# Autodesk Inventor assembly: Horizontal Weapon Assembly (Type FD)
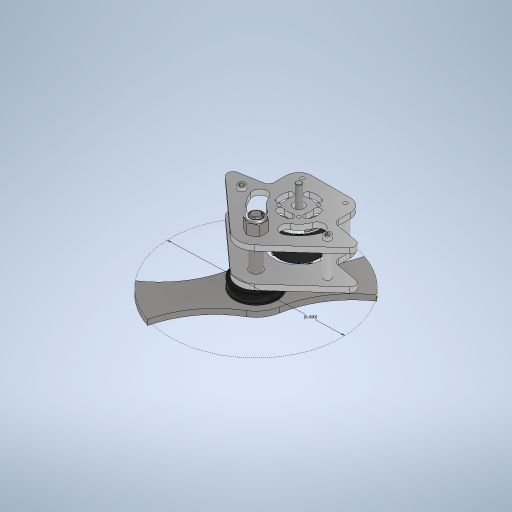
[picture p0: Inventor's stored thumbnail of the model, 512x512]
Saved by Autodesk Inventor 2023.2 (Build 272271000, 271)
## iProperties
Created: 2022-11-17
Part Number: Horizontal Weapon Assembly (Type FD)
Document SubType Name: Assembly
Designer: Nathan Cai
Mass: 397.62 g
Surface Area: 730.146 cm^2
Volume: 92.9751 cm^3
Density: 4.27663 g/cm^3
Author: Nathan Cai
## Documents named in this file (9)
- E:\Documents\Inventor\0.3rd Lawette - V3.5\Horizontal Weapon Assembly (Type FD)\Horizontal Weapon Assembly (Type FD).iam
- E:\Documents\Inventor\0.3rd Lawette - V3.5\Horizontal Weapon Assembly (Type FD)\Upright.ipt
- E:\Documents\Inventor\0.3rd Lawette - V3.5\Horizontal Weapon Assembly (Type FD)\Upright (Lower).ipt
- E:\Documents\Inventor\0.3rd Lawette - V3.5\Standoff 1in.ipt
- E:\Documents\Inventor\0.3rd Lawette - V3.5\Standoff 1.5in.ipt
- E:\Documents\Inventor\0.3rd Lawette - V3.5\Horizontal Weapon Assembly (Type FD)\90807A139_Same-Size Thread Alloy Steel Shoulder Screw.ipt
- E:\Documents\Inventor\0.3rd Lawette - V3.5\Horizontal Weapon Assembly (Type FD)\90630A121_High-Strength Steel Nylon-Insert Locknut.ipt
- E:\Documents\Inventor\0.3rd Lawette - V3.5\Horizontal Weapon Assembly (Type FD)\Weapon Stack.iam
- E:\Documents\Inventor\0.3rd Lawette - V3.5\Horizontal Weapon Assembly (Type FD)\Propdrive 3536\Propdrive V2 3536.iam
## Components (10 placed, 8 different names)
1. Upright:1 — Mate:4, Mate:5, Mate:6, Mate:7, Mate:8, Mate:9, Mate:10, Mate:11, Mate:12, Mate:13, Mate:14, Mate:16, Mate:19, Mate:20, Mate:21
2. Upright (Lower):1 — Mate:4, Mate:5, Mate:6, Flush:1, Flush:2
3. Standoff 1in:1 — Mate:7, Mate:10
4. Standoff 1in:2 — Mate:8, Mate:9
5. Standoff 1.5in:1 — Mate:11, Flush:1
6. Standoff 1.5in:2 — Mate:12, Flush:2
7. 90807A139_Same-Size Thread Alloy Steel Shoulder Screw:1 — Mate:13, Mate:14, Mate:15, Mate:17, Mate:18
8. 90630A121_High-Strength Steel Nylon-Insert Locknut:1 — Mate:15, Mate:16
9. Weapon Stack:1 [sub-assembly] — Mate:17, Mate:18
10. Propdrive V2 3536:1 [sub-assembly] — Mate:19, Mate:20, Mate:21
## Relationships (20: Mate 18, Flush 2)
- Mate:4: Upright:1 ↔ Upright (Lower):1
- Mate:5 (25.4 mm): Upright:1 ↔ Upright (Lower):1
- Mate:6: Upright:1 ↔ Upright (Lower):1
- Mate:7: Upright:1 ↔ Standoff 1in:1
- Mate:8: Upright:1 ↔ Standoff 1in:2
- Mate:9: Upright:1 ↔ Standoff 1in:2
- Mate:10: Upright:1 ↔ Standoff 1in:1
- Mate:11: Upright:1 ↔ Standoff 1.5in:1
- Mate:12: Upright:1 ↔ Standoff 1.5in:2
- Flush:1: Upright (Lower):1 ↔ Standoff 1.5in:1
- Flush:2: Upright (Lower):1 ↔ Standoff 1.5in:2
- Mate:13: Upright:1 ↔ 90807A139_Same-Size Thread Alloy Steel Shoulder Screw:1
- Mate:14: Upright:1 ↔ 90807A139_Same-Size Thread Alloy Steel Shoulder Screw:1
- Mate:15: 90807A139_Same-Size Thread Alloy Steel Shoulder Screw:1 ↔ 90630A121_High-Strength Steel Nylon-Insert Locknut:1
- Mate:16: Upright:1 ↔ 90630A121_High-Strength Steel Nylon-Insert Locknut:1
- Mate:17: 90807A139_Same-Size Thread Alloy Steel Shoulder Screw:1 ↔ Weapon Stack:1
- Mate:18: 90807A139_Same-Size Thread Alloy Steel Shoulder Screw:1 ↔ Weapon Stack:1
- Mate:19: Upright:1 ↔ Propdrive V2 3536:1
- Mate:20: Upright:1 ↔ Propdrive V2 3536:1
- Mate:21: Upright:1 ↔ Propdrive V2 3536:1
